# Autodesk Inventor assembly: Assembly1
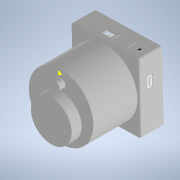
[picture p0: Inventor's stored thumbnail of the model, 180x180]
Saved by Autodesk Inventor 2020 (Build 240168000, 168)
## iProperties
Created: 2020-08-08
Part Number: Assembly1
Document SubType Name: Assembly
Designer: reide
Author: reide
## Documents named in this file (10)
- C:\Users\reide\OneDrive\Documents\Inventor\Amazon Order Button\Assembly1.iam
- C:\Users\reide\OneDrive\Documents\3d Printing\Printrbot Metal\Twisty Puzzles\I-Cubes\I-Cube Mirror Blocks 3x3x2\SS Mirror Blocks\ButtonModel.ipt
- C:\Users\reide\OneDrive\Documents\Inventor\Amazon Order Button\Button_Ring.ipt
- C:\Users\reide\OneDrive\Documents\Inventor\Amazon Order Button\Button_base.ipt
- C:\Users\reide\OneDrive\Documents\Inventor\Amazon Order Button\Marshmallow.ipt
- C:\Users\reide\OneDrive\Documents\Inventor\Amazon Order Button\Toggle_Switch.ipt
- C:\Users\reide\OneDrive\Documents\Inventor\Amazon Order Button\Base.ipt
- C:\Users\reide\OneDrive\Documents\Inventor\Amazon Order Button\Raspberry PI 3 Model A+ - Simple.ipt
- C:\Users\reide\OneDrive\Documents\Inventor\Amazon Order Button\HDMI_Cover.ipt
- C:\Users\reide\OneDrive\Documents\Inventor\Amazon Order Button\BaseBottom.ipt
## Components (9 placed, 9 different names)
1. ButtonModel:1 — Flush:1, Flush:2, Mate:1, Mate:3
2. Button_Ring:1 — Flush:1
3. Button_base:1 — Flush:2, Angle:1, Angle:2
4. Toggle_Switch:1 — Angle:1, Angle:2, Mate:2, Mate:4
5. Marshmallow:2 — Mate:1, Mate:2, Mate:3, Mate:4, Flush:3
6. Base:1 — Flush:3, Angle:3, Flush:4, Flush:5, Flush:7
7. Raspberry PI 3 Model A+ - Simple:1 — Angle:3, Flush:4, Flush:5, Flush:6
8. HDMI_Cover:1 — Flush:6
9. BaseBottom:1 — Flush:7
## Relationships (14: Flush 7, Mate 4, Angle 3)
- Flush:1: ButtonModel:1 ↔ Button_Ring:1
- Flush:2: ButtonModel:1 ↔ Button_base:1
- Angle:1 (0 deg): Button_base:1 ↔ Toggle_Switch:1
- Angle:2 (0 deg): Button_base:1 ↔ Toggle_Switch:1
- Mate:1: ButtonModel:1 ↔ Marshmallow:2
- Mate:2: Toggle_Switch:1 ↔ Marshmallow:2
- Mate:3: ButtonModel:1 ↔ Marshmallow:2
- Mate:4: Toggle_Switch:1 ↔ Marshmallow:2
- Flush:3: Marshmallow:2 ↔ Base:1
- Angle:3 (0 deg): Base:1 ↔ Raspberry PI 3 Model A+ - Simple:1
- Flush:4: Base:1 ↔ Raspberry PI 3 Model A+ - Simple:1
- Flush:5 (2 mm): Base:1 ↔ Raspberry PI 3 Model A+ - Simple:1
- Flush:6: Raspberry PI 3 Model A+ - Simple:1 ↔ HDMI_Cover:1
- Flush:7: Base:1 ↔ BaseBottom:1
